# Autodesk Inventor assembly: Planeten
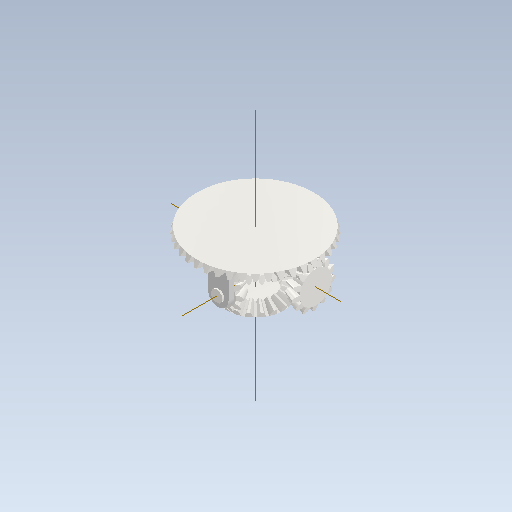
[picture p0: Inventor's stored thumbnail of the model, 512x512]
Saved by Autodesk Inventor 2021 (Build 250183000, 183)
## iProperties
Created: 2021-01-28
Part Number: Planeten
Document SubType Name: Assembly
Designer: LETPJG
Author: LETPJG
## Documents named in this file (6)
- C:\Users\LETPJG\Documents\Vault\Gruppen\Gruppe 2\Entwurf\Amphibienfahrzeug\Planeten.iam
- C:\Users\LETPJG\Documents\Vault\Gruppen\Gruppe 2\Entwurf\Amphibienfahrzeug\Planeten\Konstruktions-Assistent\Kegelräder1.iam
- C:\Users\LETPJG\Documents\Vault\Gruppen\Gruppe 2\Entwurf\Amphibienfahrzeug\Planeten\Konstruktions-Assistent\Kegelräder2.iam
- C:\Users\LETPJG\Documents\Vault\Gruppen\Gruppe 2\Entwurf\Amphibienfahrzeug\Planeten\Konstruktions-Assistent\Kegelräder15.iam
- C:\Users\LETPJG\Documents\Vault\Gruppen\Gruppe 2\Entwurf\Amphibienfahrzeug\Planeten\Konstruktions-Assistent\Kegelräder15_MIR.iam
- C:\Users\LETPJG\Documents\Vault\Gruppen\Gruppe 2\Entwurf\Amphibienfahrzeug\planetenstab.ipt
## Components (6 placed, 3 different names)
1. Kegelräder:1 [sub-assembly] — Passend:1, Passend:2, Passend:3, Passend:6, Passend:7, Passend:11
2. Kegelräder:2 [sub-assembly] — Passend:1, Passend:2, Winkel:1, Passend:9, Passend:12
3. Kegelräder:3 [sub-assembly] — Passend:3, Winkel:1, Passend:5, Passend:8, Passend:10
4. Kegelräder15_MIR:1 [sub-assembly] — Passend:5, Passend:6
5. planetenstab:1 — Passend:7, Passend:8, Passend:11
6. planetenstab:2 — Passend:9, Passend:10, Passend:12
## Relationships (12: Mate 11, Angle 1)
- Passend:1 [Mate]: Kegelräder:1 ↔ Kegelräder:2
- Passend:2 [Mate]: Kegelräder:1 ↔ Kegelräder:2
- Passend:3 [Mate]: Kegelräder:1 ↔ Kegelräder:3
- Winkel:1 [Angle] (90 deg): Kegelräder:2 ↔ Kegelräder:3
- Passend:5 [Mate]: Kegelräder:3 ↔ Kegelräder15_MIR:1
- Passend:6 [Mate] (90 mm): Kegelräder:1 ↔ Kegelräder15_MIR:1
- Passend:7 [Mate]: Kegelräder:1 ↔ planetenstab:1
- Passend:8 [Mate]: Kegelräder:3 ↔ planetenstab:1
- Passend:9 [Mate]: Kegelräder:2 ↔ planetenstab:2
- Passend:10 [Mate]: Kegelräder:3 ↔ planetenstab:2
- Passend:11 [Mate]: Kegelräder:1 ↔ planetenstab:1
- Passend:12 [Mate] (0.5 mm): Kegelräder:2 ↔ planetenstab:2
